# Autodesk Inventor assembly: INTK_017_PelletDeflectorAssembly
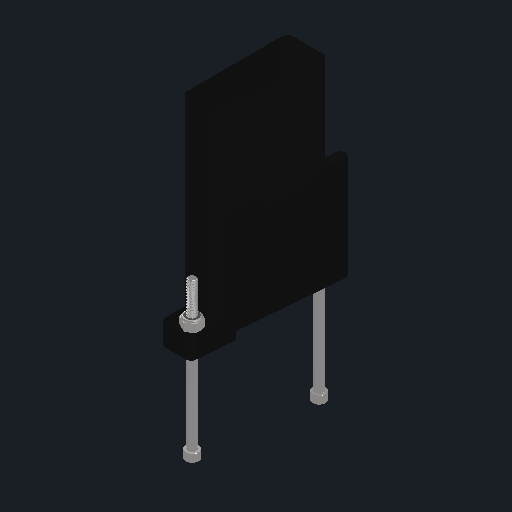
[picture p0: Inventor's stored thumbnail of the model, 512x512]
Saved by Autodesk Inventor 2024.2 (Build 282272000, 272)
## iProperties
Created: 2024-08-07
Part Number: INTK_017_PelletDeflectorAssembly
Document SubType Name: Assembly
Designer: Kenji
Mass: 227.991 g
Surface Area: 310.063 cm^2
Volume: 181.546 cm^3
Density: 1.25583 g/cm^3
Author: Kenji
## Documents named in this file (4)
- C:\Users\bobsb\OneDrive\Documents\GitHub\1622-2024-Summer-CAD-A-Thon\Intake\INTK_017_PelletDeflectorAssembly.iam
- C:\Users\bobsb\OneDrive\Documents\GitHub\1622-2024-Summer-CAD-A-Thon\Intake\INtk_016_PelletDeflector1.ipt
- C:\Users\bobsb\OneDrive\Documents\GitHub\1622-2024-Summer-CAD-A-Thon\COTS Library\Fasteners\Bolts\Socket-Head\10-32\COTS_92196A284_18-8 Stainless Steel Socket Head Screw.ipt
- C:\Users\bobsb\OneDrive\Documents\GitHub\1622-2024-Summer-CAD-A-Thon\COTS Library\Fasteners\Nuts\COTS_90631A411_10-32_Nylock_Nut.ipt
## Components (5 placed, 3 different names)
1. INtk_016_PelletDeflector1:1 — Mate:1, Mate:2, Mate:3, Mate:4, Mate:7, Mate:8
2. COTS_92196A284_18-8 Stainless Steel Socket Head Screw:1 — Mate:1, Mate:2, Mate:5
3. COTS_92196A284_18-8 Stainless Steel Socket Head Screw:2 — Mate:3, Mate:4, Mate:6
4. COTS_90631A411_10-32_Nylock_Nut:1 — Mate:5, Mate:8
5. COTS_90631A411_10-32_Nylock_Nut:2 — Mate:6, Mate:7
## Relationships (8: Mate 8)
- Mate:1: INtk_016_PelletDeflector1:1 ↔ COTS_92196A284_18-8 Stainless Steel Socket Head Screw:1
- Mate:2 (50.8254 mm): INtk_016_PelletDeflector1:1 ↔ COTS_92196A284_18-8 Stainless Steel Socket Head Screw:1
- Mate:3: INtk_016_PelletDeflector1:1 ↔ COTS_92196A284_18-8 Stainless Steel Socket Head Screw:2
- Mate:4 (58.7248 mm): INtk_016_PelletDeflector1:1 ↔ COTS_92196A284_18-8 Stainless Steel Socket Head Screw:2
- Mate:5: COTS_92196A284_18-8 Stainless Steel Socket Head Screw:1 ↔ COTS_90631A411_10-32_Nylock_Nut:1
- Mate:6: COTS_92196A284_18-8 Stainless Steel Socket Head Screw:2 ↔ COTS_90631A411_10-32_Nylock_Nut:2
- Mate:7: INtk_016_PelletDeflector1:1 ↔ COTS_90631A411_10-32_Nylock_Nut:2
- Mate:8: INtk_016_PelletDeflector1:1 ↔ COTS_90631A411_10-32_Nylock_Nut:1
